# Autodesk Inventor assembly: Extruder_assembly
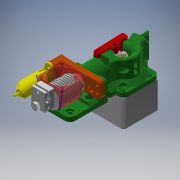
[picture p0: Inventor's stored thumbnail of the model, 180x180]
Saved by Autodesk Inventor 2016 (Build 200138000, 138)
## iProperties
Created: 2015-12-24
Part Number: Extruder_assembly
Document SubType Name: Assembly
Designer: inornate
Author: inornate
## Documents named in this file (13)
- D:\Dropbox\Soruces\3d_Print\new i3\Extruder\160119 Assembly\Extruder_assembly.iam
- D:\Dropbox\Soruces\3d_Print\new i3\Extruder\160119 Version\Extruder_mk8.ipt
- D:\Dropbox\Soruces\3d_Print\new i3\Extruder\improvement\Imported Components\Extrusor_-_Cuerpo_Extruder\TubeClamp.ipt
- D:\Dropbox\Soruces\3d_Print\new i3\Extruder\improvement\Imported Components\Extrusor_-_Cuerpo_Extruder\NEMA17.ipt
- D:\Dropbox\Soruces\3d_Print\Lincsolution\3d modeling\Imported Components\link pro\EXTRUDER_Gear_8.ipt
- D:\Dropbox\Soruces\3d_Print\new i3\Extruder\improvement\Imported Components\Extrusor_-_Tensor_Filamento\Extrusor_-_Tensor_Filamento.ipt
- D:\Dropbox\Soruces\3d_Print\new i3\Extruder\improvement\Imported Components\Extrusor_-_Cuerpo_Extruder\Bearing.ipt
- D:\Dropbox\Soruces\3d_Print\new i3\Extruder\Imported Components\E3D_V6_1.75mm_Universal_HotEnd_Mockup\E3D_V6_1.75mm_Universal_HotEnd_Mockup.ipt
- D:\Dropbox\Soruces\3d_Print\new i3\Extruder\Extruder_clamp.ipt
- D:\Dropbox\Soruces\3d_Print\new i3\Extruder\Imported Components\V6.6_Duct\V6.6_Duct.ipt
- D:\Dropbox\Soruces\3d_Print\new i3\Extruder\BLTouch.ipt
- D:\Dropbox\Soruces\3d_Print\new i3\Extruder\BLTouch_Connector.ipt
- D:\Dropbox\Soruces\3d_Print\new i3\Extruder\BLTouch_Connector_joined.ipt
## Components (12 placed, 12 different names)
1. Extruder_mk8:1 — Flush:1, Flush:2, Rigid:2, Mate:2, Cylindrical:1, Mate:4, Cylindrical:3
2. TubeClamp:1 — Flush:1
3. NEMA17:1 — Flush:2
4. EXTRUDER_Gear_8:1 — Rigid:2
5. Extrusor_-_Tensor_Filamento:1 — Mate:2, Cylindrical:1, Cylindrical:2
6. Bearing:1 — Cylindrical:2
7. E3D_V6_1.75mm_Universal_HotEnd_Mockup:1 — Mate:4, Cylindrical:3, Flush:3, Flush:4, Cylindrical:4
8. Extruder_clamp:1 — Flush:3, Cylindrical:7, Mate:6, Flush:5
9. V6.6_Duct:1 — Flush:4, Cylindrical:4
10. BLTouch:1 — Cylindrical:5, Cylindrical:6, Mate:7
11. BLTouch_Connector:1 — Cylindrical:5, Cylindrical:6, Cylindrical:7, Mate:6
12. BLTouch_Connector_joined:1 — Flush:5, Mate:7
## Relationships (17: CylindricalJoint 7, Flush 5, Mate 4, WeldJoint 1)
- Flush:1: Extruder_mk8:1 ↔ TubeClamp:1
- Flush:2: Extruder_mk8:1 ↔ NEMA17:1
- Rigid:2 [WeldJoint]: Extruder_mk8:1 ↔ EXTRUDER_Gear_8:1
- Mate:2 (0.2 mm): Extruder_mk8:1 ↔ Extrusor_-_Tensor_Filamento:1
- Cylindrical:1: Extruder_mk8:1 ↔ Extrusor_-_Tensor_Filamento:1
- Cylindrical:2: Extrusor_-_Tensor_Filamento:1 ↔ Bearing:1
- Mate:4: Extruder_mk8:1 ↔ E3D_V6_1.75mm_Universal_HotEnd_Mockup:1
- Cylindrical:3: Extruder_mk8:1 ↔ E3D_V6_1.75mm_Universal_HotEnd_Mockup:1
- Flush:3: E3D_V6_1.75mm_Universal_HotEnd_Mockup:1 ↔ Extruder_clamp:1
- Flush:4: E3D_V6_1.75mm_Universal_HotEnd_Mockup:1 ↔ V6.6_Duct:1
- Cylindrical:4: E3D_V6_1.75mm_Universal_HotEnd_Mockup:1 ↔ V6.6_Duct:1
- Cylindrical:5: BLTouch:1 ↔ BLTouch_Connector:1
- Cylindrical:6: BLTouch:1 ↔ BLTouch_Connector:1
- Cylindrical:7: Extruder_clamp:1 ↔ BLTouch_Connector:1
- Mate:6: Extruder_clamp:1 ↔ BLTouch_Connector:1
- Flush:5: Extruder_clamp:1 ↔ BLTouch_Connector_joined:1
- Mate:7: BLTouch:1 ↔ BLTouch_Connector_joined:1
